# Autodesk Inventor assembly: Montagem1
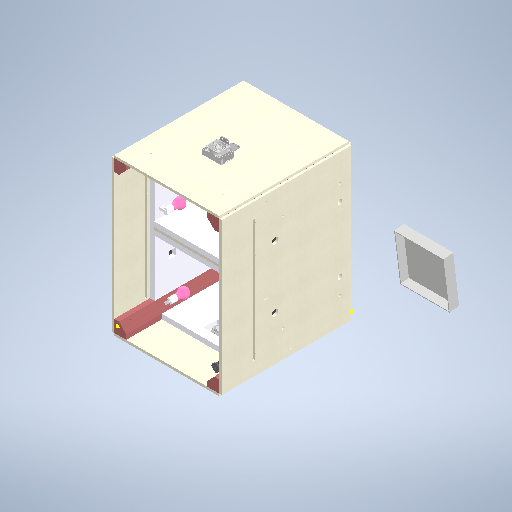
[picture p0: Inventor's stored thumbnail of the model, 512x512]
Saved by Autodesk Inventor 2025.1 (Build 291241000, 241)
## iProperties
Created: 2024-11-05
Part Number: Montagem1
Document SubType Name: Assembly
Designer: pedro
Author: pedro
## Documents named in this file (9)
- C:\Users\pedro\Documents\1-CoisasSerias\UTFPR\2024-2\Oficina\Estrutura\Montagem1.iam
- C:\Users\pedro\Documents\1-CoisasSerias\UTFPR\2024-2\Oficina\Estrutura\estrutura2.ipt
- C:\Users\pedro\Documents\1-CoisasSerias\UTFPR\2024-2\Oficina\Estrutura\Pecas Prontas\Fan\Generic 7015 axial fan simplified\Generic 7015 axial fan simplified\cooler 40x40.ipt
- C:\Users\pedro\Documents\1-CoisasSerias\UTFPR\2024-2\Oficina\Estrutura\Pecas Prontas\Let light\Soquete\Soquete para lâmpada E27 MT-2302 - DECORLUX\Soquete para lâmpada E27 MT-2302 - DECORLUX\Soquete para lâmpad.iam
- C:\Users\pedro\Documents\1-CoisasSerias\UTFPR\2024-2\Oficina\Estrutura\step mother.iam
- C:\Users\pedro\Documents\1-CoisasSerias\UTFPR\2024-2\Oficina\Estrutura\Pecas Prontas\peltier\75W Peltier Air Cooler Kit 12V (TEC1-12706) - WiMas\75W Peltier Air Cooler Kit 12V (TEC1-12706) - WiMas\75W Peltier A.iam
- C:\Users\pedro\Documents\1-CoisasSerias\UTFPR\2024-2\Oficina\Estrutura\Pecas Prontas\peltier\step\L Bracket\L Bracket\L Bracket.ipt
- C:\Users\pedro\Documents\1-CoisasSerias\UTFPR\2024-2\Oficina\Estrutura\Pecas Prontas\reservatorio.ipt
- C:\Users\pedro\Documents\1-CoisasSerias\UTFPR\2024-2\Oficina\Estrutura\Pecas Prontas\vaso.ipt
## Components (20 placed, 8 different names)
1. estrutura2:1 — Alinhado:1, Ângulo:1, Alinhado:2, Alinhado:3, Coincidente:1, Ângulo:2, Coincidente:2, Ângulo:3, Coincidente:12, Coincidente:13, Coincidente:14, Coincidente:15, Coincidente:18, Coincidente:19, Coincidente:20, Coincidente:21, Coincidente:22, Coincidente:23, Coincidente:24, Coincidente:26, Coincidente:27, Coincidente:28, Coincidente:29, Coincidente:31, Coincidente:32, Coincidente:33, Coincidente:34, Coincidente:35
2. cooler 40x40:1 — Alinhado:1, Ângulo:1, Alinhado:2, Alinhado:3
3. cooler 40x40:2
4. cooler 40x40:3
5. cooler 40x40:4
6. Soquete para lâmpad:2 [sub-assembly]
7. Soquete para lâmpad:3 [sub-assembly]
8. Soquete para lâmpad:4 [sub-assembly]
9. Soquete para lâmpad:8 [sub-assembly] — Coincidente:12, Coincidente:13
10. Soquete para lâmpad:9 [sub-assembly] — Coincidente:14, Coincidente:15
11. Soquete para lâmpad:10 [sub-assembly]
12. step mother:1 [sub-assembly] — Coincidente:18, Coincidente:19, Coincidente:20, Coincidente:21, Coincidente:22
13. step mother:3 [sub-assembly] — Coincidente:23, Coincidente:24
14. 75W Peltier A:1 [sub-assembly] — Coincidente:26, Coincidente:27
15. 75W Peltier A:2 [sub-assembly] — Coincidente:28, Coincidente:29, Coincidente:30
16. L Bracket:1 — Coincidente:30, Coincidente:31
17. L Bracket:2 — Coincidente:32
18. reservatorio:1
19. vaso:1 — Coincidente:33, Coincidente:34, Coincidente:35
20. vaso:2
## Relationships (29: Mate 23, Flush 3, Angle 3)
- Alinhado:1 [Flush] (15 mm): estrutura2:1 ↔ cooler 40x40:1
- Ângulo:1 [Angle] (0 deg): estrutura2:1 ↔ cooler 40x40:1
- Alinhado:2 [Flush] (270 mm): estrutura2:1 ↔ cooler 40x40:1
- Alinhado:3 [Flush] (310 mm): estrutura2:1 ↔ cooler 40x40:1
- Coincidente:1 [Mate]: estrutura2:1
- Ângulo:2 [Angle] (0 deg): estrutura2:1
- Coincidente:2 [Mate]: estrutura2:1
- Ângulo:3 [Angle] (0 deg): estrutura2:1
- Coincidente:12 [Mate]: estrutura2:1 ↔ Soquete para lâmpad:8
- Coincidente:13 [Mate]: estrutura2:1 ↔ Soquete para lâmpad:8
- Coincidente:14 [Mate]: estrutura2:1 ↔ Soquete para lâmpad:9
- Coincidente:15 [Mate]: estrutura2:1 ↔ Soquete para lâmpad:9
- Coincidente:18 [Mate]: estrutura2:1 ↔ step mother:1
- Coincidente:19 [Mate]: estrutura2:1 ↔ step mother:1
- Coincidente:20 [Mate]: estrutura2:1 ↔ step mother:1
- Coincidente:21 [Mate]: estrutura2:1 ↔ step mother:1
- Coincidente:22 [Mate]: estrutura2:1 ↔ step mother:1
- Coincidente:23 [Mate]: estrutura2:1 ↔ step mother:3
- Coincidente:24 [Mate]: estrutura2:1 ↔ step mother:3
- Coincidente:26 [Mate]: estrutura2:1 ↔ 75W Peltier A:1
- Coincidente:27 [Mate]: estrutura2:1 ↔ 75W Peltier A:1
- Coincidente:28 [Mate]: estrutura2:1 ↔ 75W Peltier A:2
- Coincidente:29 [Mate]: estrutura2:1 ↔ 75W Peltier A:2
- Coincidente:30 [Mate]: 75W Peltier A:2 ↔ L Bracket:1
- Coincidente:31 [Mate]: estrutura2:1 ↔ L Bracket:1
- Coincidente:32 [Mate]: estrutura2:1 ↔ L Bracket:2
- Coincidente:33 [Mate]: estrutura2:1 ↔ vaso:1
- Coincidente:34 [Mate] (192.5 mm): estrutura2:1 ↔ vaso:1
- Coincidente:35 [Mate] (97.5 mm): estrutura2:1 ↔ vaso:1
